# Autodesk Inventor assembly: led_ring_clock
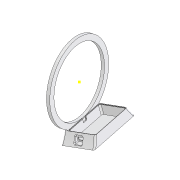
[picture p0: Inventor's stored thumbnail of the model, 180x180]
Saved by Autodesk Inventor 2020 (Build 240168000, 168)
## iProperties
Created: 2020-05-06
Part Number: led_ring_clock
Document SubType Name: Assembly
Designer: User
Author: User
## Documents named in this file (3)
- C:\Users\User\Desktop\led_ring\led_ring_clock.iam
- C:\Users\User\Desktop\led_ring\led_ring_base.ipt
- C:\Users\User\Desktop\led_ring\led_ring.ipt
## Components (2 placed, 2 different names)
1. led_ring_base:1 — Mate:1, Mate:2
2. led_ring:1 — Mate:1, Mate:2
## Relationships (2: Mate 2)
- Mate:1: led_ring_base:1 ↔ led_ring:1
- Mate:2: led_ring_base:1 ↔ led_ring:1
